# Autodesk Inventor assembly: Knife Assembly
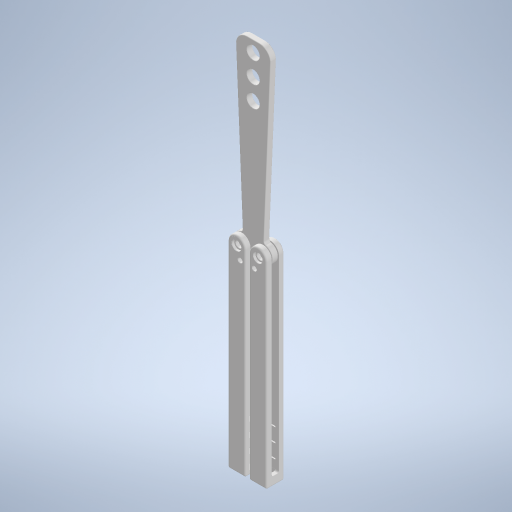
[picture p0: Inventor's stored thumbnail of the model, 512x512]
Saved by Autodesk Inventor 2023.5 (Build 275446000, 446)
## iProperties
Created: 2025-04-03
Part Number: Knife Assembly
Document SubType Name: Assembly
Designer: huy20
Author: huy20
## Documents named in this file (5)
- C:\Users\huy20\Documents\STM32\Print3D-Butterfly-Knife\SourcePart\Knife Assembly.iam
- C:\Users\huy20\Documents\STM32\Print3D-Butterfly-Knife\SourcePart\Body_Left.ipt
- C:\Users\huy20\Documents\STM32\Print3D-Butterfly-Knife\SourcePart\Body_Right.ipt
- C:\Users\huy20\Documents\STM32\Print3D-Butterfly-Knife\SourcePart\Blade.ipt
- C:\Users\huy20\Documents\Inventor\Content Center Files\R2023\en-US\ANSI B18.6.7M(02)\ANSI B18.6.7M - M3.5x0.6 x 10(6).ipt
## Components (4 placed, 4 different names)
1. Body_Right:1 — Mate:2, Mate:4, Mate:6
2. Body_Left:1 — Mate:1, Mate:3
3. Blade:1 — Mate:1, Mate:2, Mate:3, Mate:4, Mate:5
4. Square Recessed Pan Head Machine Screw - Type III - Metric M3.5x0.6 x 10:1 — Mate:5, Mate:6
## Relationships (6: Mate 6)
- Mate:1: Body_Left:1 ↔ Blade:1
- Mate:2: Body_Right:1 ↔ Blade:1
- Mate:3 (0.5015 mm): Body_Left:1 ↔ Blade:1
- Mate:4 (0.5015 mm): Body_Right:1 ↔ Blade:1
- Mate:5: Blade:1 ↔ Square Recessed Pan Head Machine Screw - Type III - Metric M3.5x0.6 x 10:1
- Mate:6: Body_Right:1 ↔ Square Recessed Pan Head Machine Screw - Type III - Metric M3.5x0.6 x 10:1
